# Autodesk Inventor assembly: Chest Assembly
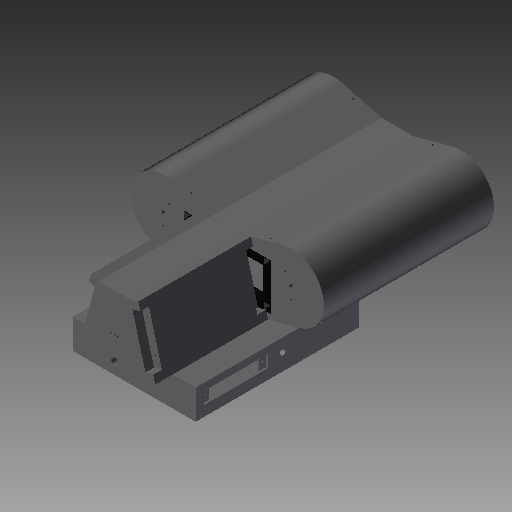
[picture p0: Inventor's stored thumbnail of the model, 512x512]
Saved by Autodesk Inventor 2017 SP1 (Build 210196100, 196)
## iProperties
Created: 2017-06-04
Part Number: Chest Assembly
Document SubType Name: Assembly
Designer: Zach
Author: Zach
## Documents named in this file (6)
- C:\Users\Zach\Documents\GitHub\tr1\src\Body\Chest Assembly\Chest Assembly.iam
- C:\Users\Zach\Documents\GitHub\tr1\src\Body\Chest Assembly\Chassis\Chassis.iam
- C:\Users\Zach\Documents\GitHub\tr1\src\Body\Chest Assembly\Backpack Assembly\Backpack.iam
- C:\Users\Zach\Documents\GitHub\tr1\src\Body\Chest Assembly\Sternum Assembly\Sternum Assembly.iam
- C:\Users\Zach\Documents\GitHub\tr1\lib\NVIDIA Jetson TK1\Jetson_TK1_FabD_3D.iam
- C:\Users\Zach\Documents\GitHub\tr1\src\Body\Chest Assembly\Torso - Solid\Torso Solid.iam
## Components (5 placed, 5 different names)
1. Chassis:1 [sub-assembly] — Flush:1, Mate:32, Mate:33
2. Backpack:1 [sub-assembly] — Mate:36, Mate:37, Mate:38, Mate:39, Mate:40, Mate:41
3. Sternum Assembly:1 [sub-assembly] — Mate:34, Mate:35, Mate:36, Mate:37, Mate:38
4. Jetson_TK1_FabD_3D:1 [sub-assembly] — Mate:39, Mate:40, Mate:41
5. Torso Solid:1 [sub-assembly] — Flush:1, Mate:32, Mate:33, Mate:34, Mate:35
## Relationships (11: Mate 10, Flush 1)
- Flush:1: Chassis:1 ↔ Torso Solid:1
- Mate:32: Chassis:1 ↔ Torso Solid:1
- Mate:33: Chassis:1 ↔ Torso Solid:1
- Mate:34: Sternum Assembly:1 ↔ Torso Solid:1
- Mate:35: Sternum Assembly:1 ↔ Torso Solid:1
- Mate:36: Backpack:1 ↔ Sternum Assembly:1
- Mate:37: Backpack:1 ↔ Sternum Assembly:1
- Mate:38: Backpack:1 ↔ Sternum Assembly:1
- Mate:39: Backpack:1 ↔ Jetson_TK1_FabD_3D:1
- Mate:40: Backpack:1 ↔ Jetson_TK1_FabD_3D:1
- Mate:41: Backpack:1 ↔ Jetson_TK1_FabD_3D:1
